# Autodesk Inventor assembly: dragonfly2CameraAndLens
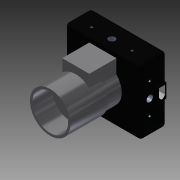
[picture p0: Inventor's stored thumbnail of the model, 180x180]
Saved by Autodesk Inventor 2013 (Build 170138000, 138)
## iProperties
Created: 2014-07-04
Part Number: dragonfly2CameraAndLens
Document SubType Name: Assembly
Designer: Nano
Author: Nano
## Documents named in this file (3)
- C:\Users\Nano\Documents\InventorByron\InventorMasterProject\panTiltSystem\dragonfly2CameraAndLens.iam
- C:\Users\Nano\Documents\InventorByron\InventorMasterProject\panTiltSystem\dragonfly2Camera.ipt
- C:\Users\Nano\Documents\InventorByron\InventorMasterProject\panTiltSystem\dragonFlyLens.ipt
## Components (2 placed, 2 different names)
1. dragonfly2Camera:1 — Flush:1, Flush:2
2. dragonFlyLens:1 — Flush:1, Flush:2
## Relationships (2: Flush 2)
- Flush:1: dragonfly2Camera:1 ↔ dragonFlyLens:1
- Flush:2: dragonfly2Camera:1 ↔ dragonFlyLens:1
